# Autodesk Inventor assembly: computer assembly
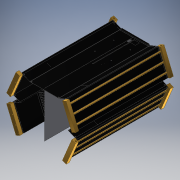
[picture p0: Inventor's stored thumbnail of the model, 180x180]
Saved by Autodesk Inventor 2018 (Build 220112000, 112)
## iProperties
Created: 2018-06-04
Part Number: computer assembly
Document SubType Name: Assembly
Designer: John Viljoen
Author: John Viljoen
## Documents named in this file (13)
- C:\Users\John Viljoen\Documents\Inventor\computer project\computer assembly.iam
- C:\Users\John Viljoen\Documents\Inventor\computer project\baseplate.ipt
- C:\Users\John Viljoen\Documents\Inventor\computer project\coverplate.ipt
- C:\Users\John Viljoen\Documents\Inventor\computer project\sideplate part 5.ipt
- C:\Users\John Viljoen\Documents\Inventor\computer project\sideplate part 4.ipt
- C:\Users\John Viljoen\Documents\Inventor\computer project\heat sink.ipt
- C:\Users\John Viljoen\Documents\Inventor\computer project\topplate.ipt
- C:\Users\John Viljoen\Documents\Inventor\computer project\sideplate part 3.ipt
- C:\Users\John Viljoen\Documents\Inventor\computer project\manifold assembly.iam
- C:\Users\John Viljoen\Documents\Inventor\computer project\manifold assembly_MIR2.iam
- C:\Users\John Viljoen\Documents\Inventor\computer project\manifold assembly_MIR3.iam
- C:\Users\John Viljoen\Documents\Inventor\computer project\my trunk assembly_MIR.iam
- C:\Users\John Viljoen\Documents\Inventor\computer project\io_shield.ipt
## Components (20 placed, 12 different names)
1. baseplate:1 — Mate:1, Flush:1, Flush:2, Mate:2, Flush:3, Flush:4, Mate:3, Flush:5, Flush:6, Mate:4, Flush:7, Flush:8, Mate:5, Mate:7, Mate:8, Flush:9, Mate:12, Mate:14, Mate:16, Mate:18, Mate:24, Mate:25, Flush:20, Mate:27, Flush:24, Flush:26, Mate:28, Mate:29, Mate:30
2. coverplate:1 — Mate:2, Flush:3, Flush:4, Mate:6, Mate:11, Flush:10, Mate:19, Flush:14, Flush:15, Flush:25
3. coverplate:2 — Mate:1, Flush:1, Flush:2, Mate:13, Flush:11, Flush:18, Flush:19
4. coverplate:3 — Mate:3, Flush:5, Flush:6, Mate:15, Flush:12, Flush:21
5. coverplate:4 — Mate:4, Flush:7, Flush:8, Mate:10, Mate:17, Flush:13, Flush:23
6. sideplate part 5:1 — Mate:5, Mate:6, Mate:7
7. sideplate part 4:1 — Mate:8, Mate:10, Flush:9
8. heat sink:1 — Mate:17, Mate:18, Flush:13
9. heat sink:2 — Mate:15, Mate:16, Flush:12
10. heat sink:3 — Mate:13, Mate:14, Flush:11
11. heat sink:4 — Mate:11, Mate:12, Flush:10
12. topplate:1 — Mate:19, Flush:14, Flush:15, Mate:20, Flush:16, Mate:21, Mate:22, Mate:23, Flush:17, Mate:26, Flush:22
13. sideplate part 3:1 — Mate:20, Flush:16, Mate:21
14. sideplate part 3:2 — Mate:22, Mate:23, Flush:17
15. manifold assembly:1 [sub-assembly] — Mate:24, Flush:18, Flush:19
16. manifold assembly:2 [sub-assembly] — Mate:25, Flush:20, Flush:21
17. manifold assembly_MIR2:1 [sub-assembly] — Mate:26, Flush:22, Flush:23
18. manifold assembly_MIR3:1 [sub-assembly] — Mate:27, Flush:24, Flush:25
19. my trunk assembly_MIR:1 [sub-assembly] — Flush:26, Mate:28, Mate:29
20. io_shield:1 — Mate:30
## Relationships (55: Mate 29, Flush 26)
- Mate:1: baseplate:1 ↔ coverplate:2
- Flush:1: baseplate:1 ↔ coverplate:2
- Flush:2: baseplate:1 ↔ coverplate:2
- Mate:2: baseplate:1 ↔ coverplate:1
- Flush:3: baseplate:1 ↔ coverplate:1
- Flush:4: baseplate:1 ↔ coverplate:1
- Mate:3: baseplate:1 ↔ coverplate:3
- Flush:5: baseplate:1 ↔ coverplate:3
- Flush:6: baseplate:1 ↔ coverplate:3
- Mate:4: baseplate:1 ↔ coverplate:4
- Flush:7: baseplate:1 ↔ coverplate:4
- Flush:8: baseplate:1 ↔ coverplate:4
- Mate:5: baseplate:1 ↔ sideplate part 5:1
- Mate:6: coverplate:1 ↔ sideplate part 5:1
- Mate:7: baseplate:1 ↔ sideplate part 5:1
- Mate:8: baseplate:1 ↔ sideplate part 4:1
- Mate:10: coverplate:4 ↔ sideplate part 4:1
- Flush:9: baseplate:1 ↔ sideplate part 4:1
- Mate:11: coverplate:1 ↔ heat sink:4
- Mate:12: baseplate:1 ↔ heat sink:4
- Flush:10: coverplate:1 ↔ heat sink:4
- Mate:13: coverplate:2 ↔ heat sink:3
- Mate:14: baseplate:1 ↔ heat sink:3
- Flush:11: coverplate:2 ↔ heat sink:3
- Mate:15: coverplate:3 ↔ heat sink:2
- Mate:16: baseplate:1 ↔ heat sink:2
- Flush:12: coverplate:3 ↔ heat sink:2
- Mate:17: coverplate:4 ↔ heat sink:1
- Mate:18: baseplate:1 ↔ heat sink:1
- Flush:13: coverplate:4 ↔ heat sink:1
- Mate:19: coverplate:1 ↔ topplate:1
- Flush:14: coverplate:1 ↔ topplate:1
- Flush:15: coverplate:1 ↔ topplate:1
- Mate:20: topplate:1 ↔ sideplate part 3:1
- Flush:16: topplate:1 ↔ sideplate part 3:1
- Mate:21: topplate:1 ↔ sideplate part 3:1
- Mate:22: topplate:1 ↔ sideplate part 3:2
- Mate:23: topplate:1 ↔ sideplate part 3:2
- Flush:17: topplate:1 ↔ sideplate part 3:2
- Mate:24: baseplate:1 ↔ manifold assembly:1
- Flush:18: coverplate:2 ↔ manifold assembly:1
- Flush:19 (-9.525 mm): coverplate:2 ↔ manifold assembly:1
- Mate:25: baseplate:1 ↔ manifold assembly:2
- Flush:20: baseplate:1 ↔ manifold assembly:2
- Flush:21 (-9.525 mm): coverplate:3 ↔ manifold assembly:2
- Mate:26: topplate:1 ↔ manifold assembly_MIR2:1
- Flush:22: topplate:1 ↔ manifold assembly_MIR2:1
- Flush:23 (-9.525 mm): coverplate:4 ↔ manifold assembly_MIR2:1
- Mate:27: baseplate:1 ↔ manifold assembly_MIR3:1
- Flush:24: baseplate:1 ↔ manifold assembly_MIR3:1
- Flush:25 (9.525 mm): coverplate:1 ↔ manifold assembly_MIR3:1
- Flush:26: baseplate:1 ↔ my trunk assembly_MIR:1
- Mate:28: baseplate:1 ↔ my trunk assembly_MIR:1
- Mate:29: baseplate:1 ↔ my trunk assembly_MIR:1
- Mate:30 (-1 mm): baseplate:1 ↔ io_shield:1
